# Autodesk Inventor assembly: RCUAssy
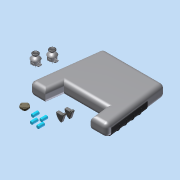
[picture p0: Inventor's stored thumbnail of the model, 180x180]
Saved by Autodesk Inventor 2011 SP1 (Build 150282100, 282)
## iProperties
Created: 2011-08-16
Part Number: RCUAssy
Document SubType Name: Assembly
Designer: dgitz
Author: dgitz
## Documents named in this file (7)
- C:\Dropbox\ICARUS\Remote Control Unit (RCU)\RCU v2\Design\RCUv2-4\RCUAssy.iam
- C:\Dropbox\ICARUS\Remote Control Unit (RCU)\RCU v2\Design\RCUv2-4\RUCBase.ipt
- C:\Dropbox\ICARUS\Remote Control Unit (RCU)\RCU v2\Design\RCUv2-4\Grip.ipt
- C:\Dropbox\ICARUS\Remote Control Unit (RCU)\RCU v2\Design\Library\XBox360DirectionalPad.ipt
- C:\Dropbox\ICARUS\Remote Control Unit (RCU)\RCU v2\Design\Library\Xbox360Button.ipt
- C:\Dropbox\ICARUS\Remote Control Unit (RCU)\RCU v2\Design\Library\Trigger.ipt
- C:\Dropbox\ICARUS\Remote Control Unit (RCU)\RCU v2\Design\Imported Components\User Library-Joystick_Asm_Left\Assembly2.iam
## Components (12 placed, 6 different names)
1. RUCBase:1 — Mate:1, Mate:2, Mate:3, Flush:1, Flush:2, Mate:4, Mate:5, Mate:6
2. Grip:1 — Mate:1, Mate:2, Mate:3
3. Grip:2 — Mate:4, Mate:5, Mate:6
4. XBox360DirectionalPad:1
5. Xbox360Button:1
6. Xbox360Button:2
7. Xbox360Button:3
8. Xbox360Button:4
9. Trigger:1
10. Trigger:2
11. Assembly2:1 [sub-assembly]
12. Assembly2:2 [sub-assembly]
## Relationships (8: Mate 6, Flush 2)
- Mate:1: RUCBase:1 ↔ Grip:1
- Mate:2: RUCBase:1 ↔ Grip:1
- Mate:3 (12.7 mm): RUCBase:1 ↔ Grip:1
- Flush:1: RUCBase:1
- Flush:2: RUCBase:1
- Mate:4: RUCBase:1 ↔ Grip:2
- Mate:5: RUCBase:1 ↔ Grip:2
- Mate:6 (12.7 mm): RUCBase:1 ↔ Grip:2
